# Autodesk Inventor assembly: Conmcept 4-Assembly
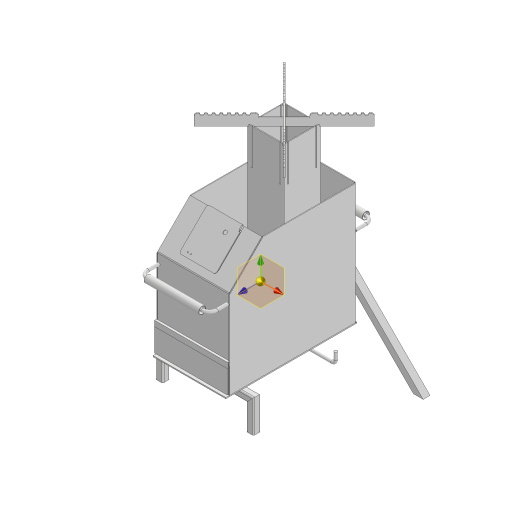
[picture p0: Inventor's stored thumbnail of the model, 512x512]
Saved by Autodesk Inventor 2024.3 (Build 283343000, 343)
## iProperties
Created: 2025-06-17
Part Number: Conmcept 4-Assembly
Document SubType Name: Assembly
Designer: ajclo
Mass: 14305.4 g
Surface Area: 18140.1 cm^2
Volume: 2029.95 cm^3
Density: 7.04719 g/cm^3
Author: ajclo
## Documents named in this file (22)
- C:\Users\ajclo\OneDrive - Stellenbosch University\Documents\BEng\Year IV\Skripsie\CAD\CAD Prototype 4\Conmcept 4-Assembly.iam
- C:\Users\ajclo\OneDrive - Stellenbosch University\Documents\BEng\Year IV\Skripsie\CAD\CAD Prototype 4\FLU-ShaftRS3.ipt
- C:\Users\ajclo\OneDrive - Stellenbosch University\Documents\BEng\Year IV\Skripsie\CAD\CAD Prototype 4\LzC-FrontPLateRS3.ipt
- C:\Users\ajclo\OneDrive - Stellenbosch University\Documents\BEng\Year IV\Skripsie\CAD\CAD Prototype 4\LzC-StoveCover.ipt
- C:\Users\ajclo\OneDrive - Stellenbosch University\Documents\BEng\Year IV\Skripsie\CAD\CAD Prototype 4\WI-ShaftRS3.ipt
- C:\Users\ajclo\OneDrive - Stellenbosch University\Documents\BEng\Year IV\Skripsie\CAD\CAD Prototype 4\BottomPlateRS3.ipt
- C:\Users\ajclo\OneDrive - Stellenbosch University\Documents\BEng\Year IV\Skripsie\CAD\CAD Prototype 4\AI-RS3.ipt
- C:\Users\ajclo\OneDrive - Stellenbosch University\Documents\BEng\Year IV\Skripsie\CAD\CAD Prototype 4\FootRS3.iam
- C:\Users\ajclo\OneDrive - Stellenbosch University\Documents\BEng\Year IV\Skripsie\CAD\CAD Prototype 4\Grid RS3.ipt
- C:\Users\ajclo\OneDrive - Stellenbosch University\Documents\BEng\Year IV\Skripsie\CAD\CAD Prototype 4\CapRS3.ipt
- C:\Users\ajclo\OneDrive - Stellenbosch University\Documents\BEng\Year IV\Skripsie\CAD\CAD Prototype 4\RS3_TubeFoot.ipt
- C:\Users\ajclo\OneDrive - Stellenbosch University\Documents\BEng\Year IV\Skripsie\CAD\CAD Prototype 4\pin.ipt
- C:\Users\ajclo\OneDrive - Stellenbosch University\Documents\BEng\Year IV\Skripsie\CAD\CAD Prototype 4\WI-Cover.ipt
- C:\Users\ajclo\OneDrive - Stellenbosch University\Documents\BEng\Year IV\Skripsie\CAD\CAD Prototype 4\AI-Cover.ipt
- C:\Users\ajclo\OneDrive - Stellenbosch University\Documents\BEng\Year IV\Skripsie\CAD\CAD Prototype 4\StoveTopAssembly.ipt.iam
- C:\Users\ajclo\OneDrive - Stellenbosch University\Documents\BEng\Year IV\Skripsie\CAD\CAD Prototype 4\GuiderailRS3.ipt
- C:\Users\ajclo\OneDrive - Stellenbosch University\Documents\BEng\Year IV\Skripsie\CAD\CAD Prototype 4\GuiderodsRS3.ipt
- C:\Users\ajclo\OneDrive - Stellenbosch University\Documents\BEng\Year IV\Skripsie\CAD\CAD Prototype 4\AllenKey-RS3.ipt
- C:\Users\ajclo\OneDrive - Stellenbosch University\Documents\BEng\Year IV\Skripsie\CAD\CAD Prototype 4\FLueExtension.ipt
- C:\Users\ajclo\OneDrive - Stellenbosch University\Documents\BEng\Year IV\Skripsie\CAD\CAD Prototype 4\Handle.ipt
- C:\Users\ajclo\OneDrive - Stellenbosch University\Documents\BEng\Year IV\Skripsie\CAD\CAD Prototype 4\Sleeve.ipt
- StoveTopAssembly.ipt
## Components (24 placed, 20 different names)
1. FLU-ShaftRS3:1 — Mate:1, Flush:1, Mate:5, Mate:6, Mate:7, Mate:10, Mate:68, Mate:69, Mate:70, Mate:71, Mate:76, Mate:77, Mate:80, Mate:90, Flush:92, Mate:91
2. LzC-FrontPLateRS3:1 — Flush:2, Mate:3, Mate:4, Mate:16, Mate:42, Mate:43, Mate:62, Mate:65, Mate:96
3. LzC-StoveCover:1 — Mate:8, Flush:3, Flush:4, Mate:11, Mate:29, Mate:30, Flush:25, Flush:93, Mate:97, Mate:98, Flush:95
4. WI-ShaftRS3:1 — Mate:1, Flush:1, Flush:2, Mate:3, Mate:4, Mate:39, Flush:21, Mate:90
5. BottomPlateRS3:1 — Mate:5, Mate:6, Mate:7, Mate:8, Flush:3, Flush:4, Mate:9, Mate:15, Mate:66, Mate:67, Flush:28
6. AI-RS3:1 — Mate:9, Mate:10, Mate:11
7. FootRS3:1 [sub-assembly] — Mate:15, Mate:16, Flush:15
8. Grid RS3:1 — Flush:28, Mate:76, Mate:77
9. RS3_TubeFoot:1 — Flush:14, Mate:29, Mate:78
10. RS3_TubeFoot:2 — Flush:14, Flush:15, Mate:30, Mate:78
11. pin:1 — Mate:39, Flush:21, Mate:41, Mate:43
12. WI-Cover:1 — Mate:41, Mate:42
13. CapRS3:1 — Mate:68, Mate:69, Mate:73, Mate:74, Mate:75
14. AI-Cover:1 — Mate:62, Mate:67
15. StoveTopAssembly.ipt:1 [sub-assembly] — Mate:81, Mate:82, Mate:83
16. GuiderailRS3:1 — Flush:25, Mate:65, Mate:66
17. GuiderodsRS3:1 — Flush:26, Flush:27, Mate:71, Mate:72
18. GuiderodsRS3:2 — Flush:26, Mate:70, Flush:27, Mate:72
19. AllenKey-RS3:1 — Mate:73, Mate:74, Mate:75
20. FLueExtension:1 — Mate:80, Mate:81, Mate:82, Mate:83, Flush:92, Mate:91
21. Handle:1 — Mate:92, Mate:93, Mate:98, Flush:94, Flush:95
22. Handle:2 — Mate:94, Mate:95, Mate:96, Flush:93, Mate:97, Flush:94
23. Sleeve:1 — Mate:94, Mate:95
24. Sleeve:2 — Mate:92, Mate:93
## Relationships (61: Mate 46, Flush 15)
- Mate:1: FLU-ShaftRS3:1 ↔ WI-ShaftRS3:1
- Flush:1: FLU-ShaftRS3:1 ↔ WI-ShaftRS3:1
- Flush:2: LzC-FrontPLateRS3:1 ↔ WI-ShaftRS3:1
- Mate:3: LzC-FrontPLateRS3:1 ↔ WI-ShaftRS3:1
- Mate:4: LzC-FrontPLateRS3:1 ↔ WI-ShaftRS3:1
- Mate:5: FLU-ShaftRS3:1 ↔ BottomPlateRS3:1
- Mate:6: FLU-ShaftRS3:1 ↔ BottomPlateRS3:1
- Mate:7: FLU-ShaftRS3:1 ↔ BottomPlateRS3:1
- Mate:8: LzC-StoveCover:1 ↔ BottomPlateRS3:1
- Flush:3: LzC-StoveCover:1 ↔ BottomPlateRS3:1
- Flush:4: LzC-StoveCover:1 ↔ BottomPlateRS3:1
- Mate:9: BottomPlateRS3:1 ↔ AI-RS3:1
- Mate:10: FLU-ShaftRS3:1 ↔ AI-RS3:1
- Mate:11: LzC-StoveCover:1 ↔ AI-RS3:1
- Mate:15: BottomPlateRS3:1 ↔ FootRS3:1
- Mate:16 (-50 mm): LzC-FrontPLateRS3:1 ↔ FootRS3:1
- Flush:14: RS3_TubeFoot:1 ↔ RS3_TubeFoot:2
- Mate:29: LzC-StoveCover:1 ↔ RS3_TubeFoot:1
- Flush:15: FootRS3:1 ↔ RS3_TubeFoot:2
- Mate:30 (-100 mm): LzC-StoveCover:1 ↔ RS3_TubeFoot:2
- Mate:39: WI-ShaftRS3:1 ↔ pin:1
- Flush:21: WI-ShaftRS3:1 ↔ pin:1
- Mate:41: pin:1 ↔ WI-Cover:1
- Mate:42 (1 mm): LzC-FrontPLateRS3:1 ↔ WI-Cover:1
- Mate:43 (73.6 mm): LzC-FrontPLateRS3:1 ↔ pin:1
- Mate:62: LzC-FrontPLateRS3:1 ↔ AI-Cover:1
- Flush:25: LzC-StoveCover:1 ↔ GuiderailRS3:1
- Mate:65: LzC-FrontPLateRS3:1 ↔ GuiderailRS3:1
- Mate:66 (80 mm): BottomPlateRS3:1 ↔ GuiderailRS3:1
- Mate:67: BottomPlateRS3:1 ↔ AI-Cover:1
- Mate:68: FLU-ShaftRS3:1 ↔ CapRS3:1
- Mate:69: FLU-ShaftRS3:1 ↔ CapRS3:1
- Flush:26: GuiderodsRS3:1 ↔ GuiderodsRS3:2
- Mate:70 (-13 mm): FLU-ShaftRS3:1 ↔ GuiderodsRS3:2
- Flush:27: GuiderodsRS3:1 ↔ GuiderodsRS3:2
- Mate:71: FLU-ShaftRS3:1 ↔ GuiderodsRS3:1
- Mate:72 (50 mm): GuiderodsRS3:1 ↔ GuiderodsRS3:2
- Mate:73: CapRS3:1 ↔ AllenKey-RS3:1
- Mate:74: CapRS3:1 ↔ AllenKey-RS3:1
- Mate:75 (44.5 mm): CapRS3:1 ↔ AllenKey-RS3:1
- Flush:28: BottomPlateRS3:1 ↔ Grid RS3:1
- Mate:76: FLU-ShaftRS3:1 ↔ Grid RS3:1
- Mate:77: FLU-ShaftRS3:1 ↔ Grid RS3:1
- Mate:78: RS3_TubeFoot:1 ↔ RS3_TubeFoot:2
- Mate:80: FLU-ShaftRS3:1 ↔ FLueExtension:1
- Mate:81: StoveTopAssembly.ipt:1 ↔ FLueExtension:1
- Mate:82: StoveTopAssembly.ipt:1 ↔ FLueExtension:1
- Mate:83: StoveTopAssembly.ipt:1 ↔ FLueExtension:1
- Mate:90: FLU-ShaftRS3:1 ↔ WI-ShaftRS3:1
- Flush:92: FLU-ShaftRS3:1 ↔ FLueExtension:1
- Mate:91: FLU-ShaftRS3:1 ↔ FLueExtension:1
- Mate:92: Handle:1 ↔ Sleeve:2
- Mate:93: Handle:1 ↔ Sleeve:2
- Mate:94: Handle:2 ↔ Sleeve:1
- Mate:95: Handle:2 ↔ Sleeve:1
- Mate:96: LzC-FrontPLateRS3:1 ↔ Handle:2
- Flush:93 (1 mm): LzC-StoveCover:1 ↔ Handle:2
- Mate:97 (-120 mm): LzC-StoveCover:1 ↔ Handle:2
- Mate:98: LzC-StoveCover:1 ↔ Handle:1
- Flush:94: Handle:1 ↔ Handle:2
- Flush:95 (112 mm): LzC-StoveCover:1 ↔ Handle:1
